# Autodesk Inventor assembly: HopperAssembly
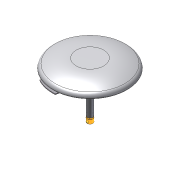
[picture p0: Inventor's stored thumbnail of the model, 180x180]
Saved by Autodesk Inventor 2012 (Build 160160000, 160)
## iProperties
Created: 2013-01-22
Part Number: HopperAssembly
Document SubType Name: Assembly
Designer: JesseK
Mass: 736.339 g
Surface Area: 9766.65 cm^2
Volume: 1935.7 cm^3
Density: 0.380399 g/cm^3
Author: JesseK
## Documents named in this file (7)
- Z:\UserData\Documents\Inventor\team1885frc\Robot2013\Hopper\HopperAssembly.iam
- Z:\UserData\Documents\Inventor\team1885frc\Robot2013\Hopper\HopperBucket.ipt
- Z:\UserData\Documents\Inventor\team1885frc\Robot2013\Hopper\HopperPlate.ipt
- Z:\UserData\Documents\Inventor\team1885frc\Robot2013\Hopper\HopperCylinderMount.ipt
- Z:\UserData\Documents\Inventor\team1885frc\Pneumatics\043-5_DQ_3-5inStrokex075\043_5_DQ_F_D_166_3_.iam
- Z:\UserData\Documents\Inventor\team1885frc\Pneumatics\043-5_DQ_3-5inStrokex075\D_9.ipt
- Z:\UserData\Documents\Inventor\team1885frc\Robot2013\Game\disc.ipt
## Components (9 placed, 6 different names)
1. HopperBucket:1 — Mate:1, Mate:2, Flush:1
2. HopperPlate:1 — Mate:1, Mate:8, Flush:2, Mate:14
3. HopperCylinderMount:1 — Mate:2, Flush:1, Mate:5, Mate:12, Mate:13
4. D-9:1 — Mate:5
5. disc:1 — Mate:8, Flush:2, Mate:9, Flush:3
6. disc:2 — Mate:10, Mate:11, Flush:4, Flush:5
7. disc:3 — Mate:9, Mate:10, Flush:3, Flush:4
8. disc:4 — Mate:11, Flush:5
9. 043.5-DQ:1 [sub-assembly] — Mate:12, Mate:13, Mate:14
## Relationships (15: Mate 10, Flush 5)
- Mate:1: HopperBucket:1 ↔ HopperPlate:1
- Mate:2: HopperBucket:1 ↔ HopperCylinderMount:1
- Flush:1: HopperBucket:1 ↔ HopperCylinderMount:1
- Mate:5: HopperCylinderMount:1 ↔ D-9:1
- Mate:8: HopperPlate:1 ↔ disc:1
- Flush:2 (12.7 mm): HopperPlate:1 ↔ disc:1
- Mate:9: disc:1 ↔ disc:3
- Mate:10: disc:2 ↔ disc:3
- Mate:11: disc:2 ↔ disc:4
- Flush:3 (12.7 mm): disc:1 ↔ disc:3
- Flush:4 (12.7 mm): disc:2 ↔ disc:3
- Flush:5 (12.7 mm): disc:2 ↔ disc:4
- Mate:12: HopperCylinderMount:1 ↔ 043.5-DQ:1
- Mate:13: HopperCylinderMount:1 ↔ 043.5-DQ:1
- Mate:14 (6.35 mm): HopperPlate:1 ↔ 043.5-DQ:1
